# Autodesk Inventor assembly: 下部分
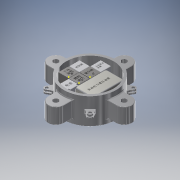
[picture p0: Inventor's stored thumbnail of the model, 180x180]
Saved by Autodesk Inventor 2018.3 (Build 223284000, 284)
## iProperties
Created: 2018-12-27
Part Number: 下部分
Material: 常规
Document SubType Name: Assembly
Designer: 丁子鸣
Author: 丁子鸣
## Documents named in this file (6)
- C:\Users\丁子鸣\Desktop\比赛图\下部分.iam
- C:\Users\丁子鸣\Desktop\比赛图\下底盘.ipt
- C:\Users\丁子鸣\Desktop\比赛图\发动机&液压泵.ipt
- C:\Users\丁子鸣\Desktop\比赛图\电池.ipt
- C:\Users\丁子鸣\Desktop\比赛图\工作油&燃油&氧化物.ipt
- C:\Users\丁子鸣\Desktop\比赛图\冷却滤油装置&控制阀.ipt
## Components (8 placed, 5 different names)
1. 下底盘:1 — 配合:1, 配合:2, 配合:3, 配合:4, 配合:5, 配合:6, 配合:7
2. 发动机&液压泵:1 — 配合:1
3. 电池:1 — 配合:2
4. 工作油&燃油&氧化物:1 — 配合:3
5. 工作油&燃油&氧化物:2 — 配合:5
6. 工作油&燃油&氧化物:3 — 配合:6
7. 冷却滤油装置&控制阀:1 — 配合:7
8. 冷却滤油装置&控制阀:2 — 配合:4
## Relationships (7: Mate 7)
- 配合:1 [Mate]: 下底盘:1 ↔ 发动机&液压泵:1
- 配合:2 [Mate]: 下底盘:1 ↔ 电池:1
- 配合:3 [Mate]: 下底盘:1 ↔ 工作油&燃油&氧化物:1
- 配合:4 [Mate]: 下底盘:1 ↔ 冷却滤油装置&控制阀:2
- 配合:5 [Mate]: 下底盘:1 ↔ 工作油&燃油&氧化物:2
- 配合:6 [Mate]: 下底盘:1 ↔ 工作油&燃油&氧化物:3
- 配合:7 [Mate]: 下底盘:1 ↔ 冷却滤油装置&控制阀:1
